# Autodesk Inventor assembly: Assembly1
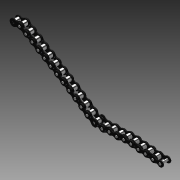
[picture p0: Inventor's stored thumbnail of the model, 180x180]
Saved by Autodesk Inventor 2011 (Build 150239000, 239)
## iProperties
Created: 2011-01-19
Part Number: Assembly1
Document SubType Name: Assembly
Designer: fcboe
Author: fcboe
## Documents named in this file (3)
- C:\Users\fcboe\Desktop\Assembly1.iam
- C:\Users\fcboe\Desktop\Robotics\Drive Train Parts\Chain#35RollLink_Easternbearings_PEEC35RIV.ipt
- C:\Users\fcboe\Desktop\Robotics\Drive Train Parts\Chain#35PinLink_Easternbearings_PEEC35RIV.ipt
## Components (22 placed, 2 different names)
1. Chain#35RollLink_Easternbearings_PEEC35RIV:1 — Insert:16
2. Chain#35RollLink_Easternbearings_PEEC35RIV:2 — Insert:7, Insert:8
3. Chain#35RollLink_Easternbearings_PEEC35RIV:3 — Insert:11, Insert:12
4. Chain#35RollLink_Easternbearings_PEEC35RIV:4 — Insert:15, Insert:17
5. Chain#35RollLink_Easternbearings_PEEC35RIV:5 — Insert:18, Insert:19
6. Chain#35RollLink_Easternbearings_PEEC35RIV:6 — Insert:20, Insert:21
7. Chain#35RollLink_Easternbearings_PEEC35RIV:11 — Insert:13, Insert:14
8. Chain#35RollLink_Easternbearings_PEEC35RIV:12 — Insert:9, Insert:10
9. Chain#35RollLink_Easternbearings_PEEC35RIV:13 — Insert:5, Insert:6
10. Chain#35RollLink_Easternbearings_PEEC35RIV:14 — Insert:3, Insert:4
11. Chain#35RollLink_Easternbearings_PEEC35RIV:15 — Insert:1, Insert:2
12. Chain#35PinLink_Easternbearings_PEEC35RIV:1 — Insert:1, Insert:16
13. Chain#35PinLink_Easternbearings_PEEC35RIV:2 — Insert:2, Insert:3
14. Chain#35PinLink_Easternbearings_PEEC35RIV:3 — Insert:4, Insert:5
15. Chain#35PinLink_Easternbearings_PEEC35RIV:4 — Insert:6, Insert:7
16. Chain#35PinLink_Easternbearings_PEEC35RIV:5 — Insert:8, Insert:9
17. Chain#35PinLink_Easternbearings_PEEC35RIV:6 — Insert:10, Insert:11
18. Chain#35PinLink_Easternbearings_PEEC35RIV:7 — Insert:12, Insert:13
19. Chain#35PinLink_Easternbearings_PEEC35RIV:8 — Insert:14, Insert:15
20. Chain#35PinLink_Easternbearings_PEEC35RIV:9 — Insert:17, Insert:18
21. Chain#35PinLink_Easternbearings_PEEC35RIV:10 — Insert:21
22. Chain#35PinLink_Easternbearings_PEEC35RIV:17 — Insert:19, Insert:20
## Relationships (21: Insert 21)
- Insert:1: Chain#35RollLink_Easternbearings_PEEC35RIV:15 ↔ Chain#35PinLink_Easternbearings_PEEC35RIV:1
- Insert:2: Chain#35RollLink_Easternbearings_PEEC35RIV:15 ↔ Chain#35PinLink_Easternbearings_PEEC35RIV:2
- Insert:3: Chain#35RollLink_Easternbearings_PEEC35RIV:14 ↔ Chain#35PinLink_Easternbearings_PEEC35RIV:2
- Insert:4: Chain#35RollLink_Easternbearings_PEEC35RIV:14 ↔ Chain#35PinLink_Easternbearings_PEEC35RIV:3
- Insert:5: Chain#35RollLink_Easternbearings_PEEC35RIV:13 ↔ Chain#35PinLink_Easternbearings_PEEC35RIV:3
- Insert:6: Chain#35RollLink_Easternbearings_PEEC35RIV:13 ↔ Chain#35PinLink_Easternbearings_PEEC35RIV:4
- Insert:7: Chain#35RollLink_Easternbearings_PEEC35RIV:2 ↔ Chain#35PinLink_Easternbearings_PEEC35RIV:4
- Insert:8: Chain#35RollLink_Easternbearings_PEEC35RIV:2 ↔ Chain#35PinLink_Easternbearings_PEEC35RIV:5
- Insert:9: Chain#35RollLink_Easternbearings_PEEC35RIV:12 ↔ Chain#35PinLink_Easternbearings_PEEC35RIV:5
- Insert:10: Chain#35RollLink_Easternbearings_PEEC35RIV:12 ↔ Chain#35PinLink_Easternbearings_PEEC35RIV:6
- Insert:11: Chain#35RollLink_Easternbearings_PEEC35RIV:3 ↔ Chain#35PinLink_Easternbearings_PEEC35RIV:6
- Insert:12: Chain#35RollLink_Easternbearings_PEEC35RIV:3 ↔ Chain#35PinLink_Easternbearings_PEEC35RIV:7
- Insert:13: Chain#35RollLink_Easternbearings_PEEC35RIV:11 ↔ Chain#35PinLink_Easternbearings_PEEC35RIV:7
- Insert:14: Chain#35RollLink_Easternbearings_PEEC35RIV:11 ↔ Chain#35PinLink_Easternbearings_PEEC35RIV:8
- Insert:15: Chain#35RollLink_Easternbearings_PEEC35RIV:4 ↔ Chain#35PinLink_Easternbearings_PEEC35RIV:8
- Insert:16: Chain#35RollLink_Easternbearings_PEEC35RIV:1 ↔ Chain#35PinLink_Easternbearings_PEEC35RIV:1
- Insert:17: Chain#35RollLink_Easternbearings_PEEC35RIV:4 ↔ Chain#35PinLink_Easternbearings_PEEC35RIV:9
- Insert:18: Chain#35RollLink_Easternbearings_PEEC35RIV:5 ↔ Chain#35PinLink_Easternbearings_PEEC35RIV:9
- Insert:19: Chain#35RollLink_Easternbearings_PEEC35RIV:5 ↔ Chain#35PinLink_Easternbearings_PEEC35RIV:17
- Insert:20: Chain#35RollLink_Easternbearings_PEEC35RIV:6 ↔ Chain#35PinLink_Easternbearings_PEEC35RIV:17
- Insert:21: Chain#35RollLink_Easternbearings_PEEC35RIV:6 ↔ Chain#35PinLink_Easternbearings_PEEC35RIV:10
